# Autodesk Inventor assembly: ArmAssemblyTest
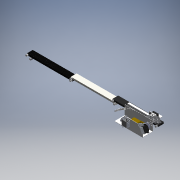
[picture p0: Inventor's stored thumbnail of the model, 180x180]
Saved by Autodesk Inventor 2019 (Build 230136000, 136)
## iProperties
Created: 2019-01-29
Part Number: ArmAssemblyTest
Document SubType Name: Assembly
Designer: User
Mass: 2383.53 g
Surface Area: 4026.03 cm^2
Volume: 987.084 cm^3
Density: 2.41472 g/cm^3
Author: User
## Documents named in this file (6)
- C:\Robotics\CAD\2018-19_CAD\Collection\ArmAssemblyTest.iam
- C:\Robotics\CAD\2018-19_CAD\Collection\sorterbucket.iam
- C:\Robotics\CAD\2018-19_CAD\Collection\slide to axle bracet.ipt
- C:\Robotics\CAD\2018-19_CAD\Collection\Lift2.iam
- C:\Robotics\CAD\2018-19_CAD\bucket hlder.ipt
- C:\Robotics\CAD\2018-19_CAD\Field Pieces\Gold.ipt
## Components (6 placed, 5 different names)
1. sorterbucket:1 [sub-assembly] — Flush:3, Mate:2, Flush:4, Angle:1, Mate:6, Mate:8, Flush:8
2. slide to axle bracet:1 — Mate:3, Flush:5, Flush:6, Mate:4, Mate:5
3. Lift2:1 [sub-assembly] — Mate:1, Flush:1, Flush:2, Mate:3, Flush:5, Flush:6, Angle:2
4. bucket hlder:1 — Mate:1, Flush:1, Flush:2, Flush:3, Mate:2, Flush:4, Angle:1
5. Gold:1 — Mate:7, Flush:7, Mate:8
6. Gold:2 — Mate:6, Mate:7, Flush:7, Flush:8
## Relationships (18: Mate 8, Flush 8, Angle 2)
- Mate:1: Lift2:1 ↔ bucket hlder:1
- Flush:1 (-14.986 mm): Lift2:1 ↔ bucket hlder:1
- Flush:2 (25.4 mm): Lift2:1 ↔ bucket hlder:1
- Flush:3: sorterbucket:1 ↔ bucket hlder:1
- Mate:2: sorterbucket:1 ↔ bucket hlder:1
- Flush:4 (-32.0802 mm): sorterbucket:1 ↔ bucket hlder:1
- Mate:3: slide to axle bracet:1 ↔ Lift2:1
- Flush:5 (22.606 mm): slide to axle bracet:1 ↔ Lift2:1
- Flush:6 (13.081 mm): slide to axle bracet:1 ↔ Lift2:1
- Mate:4: slide to axle bracet:1
- Mate:5: slide to axle bracet:1
- Angle:1 (0 deg): sorterbucket:1 ↔ bucket hlder:1
- Angle:2 (90 deg): Lift2:1
- Mate:6: sorterbucket:1 ↔ Gold:2
- Mate:7: Gold:1 ↔ Gold:2
- Flush:7: Gold:1 ↔ Gold:2
- Mate:8: sorterbucket:1 ↔ Gold:1
- Flush:8 (101.6 mm): sorterbucket:1 ↔ Gold:2
